# Autodesk Inventor assembly: MG-Powerboard
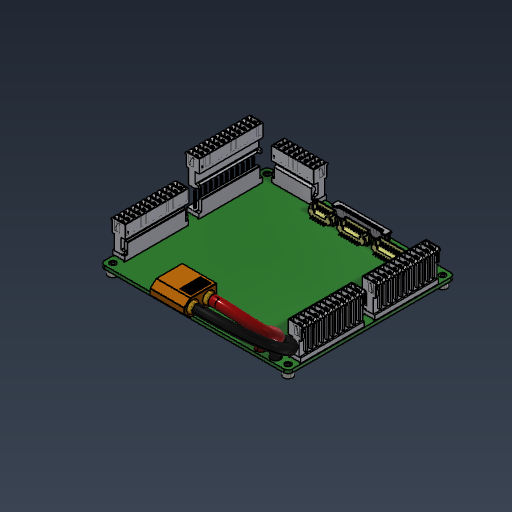
[picture p0: Inventor's stored thumbnail of the model, 512x512]
Saved by Autodesk Inventor 2023.1 (Build 271208000, 208)
## iProperties
Part Number: MG-Powerboard
Material: Generisch
Document SubType Name: Assembly
Designer: rYan
Mass: 22.1221 g
Surface Area: 374.509 cm^2
Volume: 22.3452 cm^3
Density: 0.990013 g/cm^3
Author: rYan
## Documents named in this file (14)
- D:\TIGERsGIT\Hardware\mechanik\2024\Inventor\Robot\Electronics\MG-Powerboard.iam
- D:\TIGERsGIT\Hardware\mechanik\2024\Inventor\Robot\Electronics\Powerboard.ipt
- D:\TIGERsGIT\Hardware\mechanik\2024\Inventor\Purchased Parts\MTA100 8pin Connector Straight.ipt
- D:\TIGERsGIT\Hardware\mechanik\2024\Inventor\Purchased Parts\MTA100 8pin AWG24 polarized.ipt
- D:\TIGERsGIT\Hardware\mechanik\2024\Inventor\Purchased Parts\MTA100 12pin Connector Straight.ipt
- D:\TIGERsGIT\Hardware\mechanik\2024\Inventor\Purchased Parts\MTA100 12pin AWG24 polarized.ipt
- D:\TIGERsGIT\Hardware\mechanik\2024\Inventor\Purchased Parts\XT60 Stecker.ipt
- D:\TIGERsGIT\Hardware\mechanik\2024\Inventor\Robot\Electronics\MG-Powerboard\AIP\Kabel und Kabelbaum\MG-Powerboard.Kabelbaum.iam
- D:\TIGERsGIT\Hardware\mechanik\2024\Inventor\Purchased Parts\Micro-USB.ipt
- D:\TIGERsGIT\Hardware\mechanik\2024\Inventor\Purchased Parts\TE FFC Con 40pin 0.5mm vertical.ipt
- D:\TIGERsGIT\Hardware\mechanik\2024\Inventor\Purchased Parts\DF13C-8P-1.25V.ipt
- D:\TIGERsGIT\Hardware\mechanik\2024\Inventor\Purchased Parts\DF13C-6P-1.25V.ipt
- D:\TIGERsGIT\Hardware\mechanik\2024\Inventor\Purchased Parts\DF13C-12P-1.25V.ipt
- D:\TIGERsGIT\Hardware\mechanik\2024\Inventor\Purchased Parts\Spacer M2 3mm.ipt
## Components (22 placed, 13 different names)
1. Powerboard:1 — Fluchtend:1, Fluchtend:2, Fluchtend:3, Tangential:5, Tangential:6, Tangential:7, Tangential:8, Fluchtend:20, Fluchtend:21, Fluchtend:22, Fluchtend:23, Fluchtend:24, Fluchtend:25, Fluchtend:26, Fluchtend:27, Tangential:10, Fluchtend:36, Fluchtend:37, Passend:15, Passend:16, Passend:18, Fluchtend:47, Passend:21, Passend:22, Passend:23, Passend:24, Passend:25, Einfügen:1, Einfügen:2, Einfügen:3, Einfügen:4
2. MTA100 12pin Connector Straight:1 — Tangential:6, Fluchtend:22, Fluchtend:27, Fluchtend:30, Fluchtend:31, Passend:7
3. MTA100 12pin Connector Straight:2 — Tangential:5, Fluchtend:23, Fluchtend:26, Fluchtend:28, Fluchtend:29, Passend:8
4. MTA100 12pin Connector Straight:3 — Tangential:7, Fluchtend:21, Fluchtend:25, Fluchtend:32, Fluchtend:34, Passend:6
5. MTA100 12pin Connector Straight:4 — Tangential:8, Fluchtend:20, Fluchtend:24, Fluchtend:33, Fluchtend:35, Passend:5, Passend:26
6. MTA100 12pin AWG24 polarized:1 — Fluchtend:30, Fluchtend:31, Passend:7
7. MTA100 12pin AWG24 polarized:2 — Fluchtend:28, Fluchtend:29, Passend:8
8. MTA100 12pin AWG24 polarized:3 — Fluchtend:33, Fluchtend:35, Passend:5, Passend:26
9. MTA100 12pin AWG24 polarized:4 — Fluchtend:32, Fluchtend:34, Passend:6
10. MTA100 8pin Connector Straight:1 — Tangential:10, Fluchtend:36, Fluchtend:37, Passend:9, Fluchtend:38, Fluchtend:39
11. MTA100 AWG24 8pin polarized:1 — Passend:9, Fluchtend:38, Fluchtend:39
12. XT60 Stecker:1 — Passend:15, Passend:16
13. MG-Powerboard.Kabelbaum [sub-assembly]
14. Micro-USB 47346-0001:1 — Passend:18, Fluchtend:47, Passend:21
15. TE FFC Con 40pin 0.5mm vertical:1 — Passend:22, Fluchtend:50
16. DF13C-8P-1.25V:1 — Passend:23, Fluchtend:55, Fluchtend:56
17. DF13C-6P-1.25V:1 — Passend:24, Fluchtend:53, Fluchtend:54
18. DF13C-12P-1.25V:1 — Passend:25, Fluchtend:51, Fluchtend:52
19. Spacer M2 3mm:1 — Einfügen:2
20. Spacer M2 3mm:2 — Einfügen:1
21. Spacer M2 3mm:3 — Einfügen:4
22. Spacer M2 3mm:4 — Einfügen:3
## Relationships (54: Flush 31, Mate 14, Tangent 5, Insert 4)
- Fluchtend:1 [Flush]: Powerboard:1
- Fluchtend:2 [Flush]: Powerboard:1
- Fluchtend:3 [Flush]: Powerboard:1
- Tangential:5: Powerboard:1 ↔ MTA100 12pin Connector Straight:2
- Tangential:6: Powerboard:1 ↔ MTA100 12pin Connector Straight:1
- Tangential:7: Powerboard:1 ↔ MTA100 12pin Connector Straight:3
- Tangential:8: Powerboard:1 ↔ MTA100 12pin Connector Straight:4
- Fluchtend:20 [Flush]: Powerboard:1 ↔ MTA100 12pin Connector Straight:4
- Fluchtend:21 [Flush]: Powerboard:1 ↔ MTA100 12pin Connector Straight:3
- Fluchtend:22 [Flush]: Powerboard:1 ↔ MTA100 12pin Connector Straight:1
- Fluchtend:23 [Flush]: Powerboard:1 ↔ MTA100 12pin Connector Straight:2
- Fluchtend:24 [Flush] (8 mm): Powerboard:1 ↔ MTA100 12pin Connector Straight:4
- Fluchtend:25 [Flush] (6 mm): Powerboard:1 ↔ MTA100 12pin Connector Straight:3
- Fluchtend:26 [Flush] (6 mm): Powerboard:1 ↔ MTA100 12pin Connector Straight:2
- Fluchtend:27 [Flush] (8 mm): Powerboard:1 ↔ MTA100 12pin Connector Straight:1
- Fluchtend:28 [Flush]: MTA100 12pin Connector Straight:2 ↔ MTA100 12pin AWG24 polarized:2
- Fluchtend:29 [Flush] (-0.3 mm): MTA100 12pin Connector Straight:2 ↔ MTA100 12pin AWG24 polarized:2
- Fluchtend:30 [Flush]: MTA100 12pin Connector Straight:1 ↔ MTA100 12pin AWG24 polarized:1
- Fluchtend:31 [Flush] (-0.3 mm): MTA100 12pin Connector Straight:1 ↔ MTA100 12pin AWG24 polarized:1
- Fluchtend:32 [Flush]: MTA100 12pin Connector Straight:3 ↔ MTA100 12pin AWG24 polarized:4
- Fluchtend:33 [Flush]: MTA100 12pin Connector Straight:4 ↔ MTA100 12pin AWG24 polarized:3
- Fluchtend:34 [Flush] (-0.3 mm): MTA100 12pin Connector Straight:3 ↔ MTA100 12pin AWG24 polarized:4
- Fluchtend:35 [Flush] (-0.3 mm): MTA100 12pin Connector Straight:4 ↔ MTA100 12pin AWG24 polarized:3
- Passend:5 [Mate]: MTA100 12pin Connector Straight:4 ↔ MTA100 12pin AWG24 polarized:3
- Passend:6 [Mate]: MTA100 12pin Connector Straight:3 ↔ MTA100 12pin AWG24 polarized:4
- Passend:7 [Mate]: MTA100 12pin Connector Straight:1 ↔ MTA100 12pin AWG24 polarized:1
- Passend:8 [Mate]: MTA100 12pin Connector Straight:2 ↔ MTA100 12pin AWG24 polarized:2
- Tangential:10: Powerboard:1 ↔ MTA100 8pin Connector Straight:1
- Fluchtend:36 [Flush]: Powerboard:1 ↔ MTA100 8pin Connector Straight:1
- Fluchtend:37 [Flush] (8 mm): Powerboard:1 ↔ MTA100 8pin Connector Straight:1
- Passend:9 [Mate]: MTA100 8pin Connector Straight:1 ↔ MTA100 AWG24 8pin polarized:1
- Fluchtend:38 [Flush]: MTA100 8pin Connector Straight:1 ↔ MTA100 AWG24 8pin polarized:1
- Fluchtend:39 [Flush] (-0.2 mm): MTA100 8pin Connector Straight:1 ↔ MTA100 AWG24 8pin polarized:1
- Passend:15 [Mate] (34.6 mm): Powerboard:1 ↔ XT60 Stecker:1
- Passend:16 [Mate] (23 mm): Powerboard:1 ↔ XT60 Stecker:1
- Passend:18 [Mate]: Powerboard:1 ↔ Micro-USB 47346-0001:1
- Fluchtend:47 [Flush]: Powerboard:1 ↔ Micro-USB 47346-0001:1
- Passend:21 [Mate] (32 mm): Powerboard:1 ↔ Micro-USB 47346-0001:1
- Passend:22 [Mate]: Powerboard:1 ↔ TE FFC Con 40pin 0.5mm vertical:1
- Fluchtend:50 [Flush] (-3 mm): TE FFC Con 40pin 0.5mm vertical:1
- Passend:23 [Mate]: Powerboard:1 ↔ DF13C-8P-1.25V:1
- Passend:24 [Mate]: Powerboard:1 ↔ DF13C-6P-1.25V:1
- Passend:25 [Mate]: Powerboard:1 ↔ DF13C-12P-1.25V:1
- Fluchtend:51 [Flush] (24 mm): DF13C-12P-1.25V:1
- Fluchtend:52 [Flush] (33 mm): DF13C-12P-1.25V:1
- Fluchtend:53 [Flush] (10 mm): DF13C-6P-1.25V:1
- Fluchtend:54 [Flush] (-33 mm): DF13C-6P-1.25V:1
- Fluchtend:55 [Flush] (-5 mm): DF13C-8P-1.25V:1
- Fluchtend:56 [Flush] (-33 mm): DF13C-8P-1.25V:1
- Passend:26 [Mate] (2 mm): MTA100 12pin Connector Straight:4 ↔ MTA100 12pin AWG24 polarized:3
- Einfügen:1 [Insert]: Powerboard:1 ↔ Spacer M2 3mm:2
- Einfügen:2 [Insert]: Powerboard:1 ↔ Spacer M2 3mm:1
- Einfügen:3 [Insert]: Powerboard:1 ↔ Spacer M2 3mm:4
- Einfügen:4 [Insert]: Powerboard:1 ↔ Spacer M2 3mm:3
